# Autodesk Inventor assembly: RollerAssemblyBearing
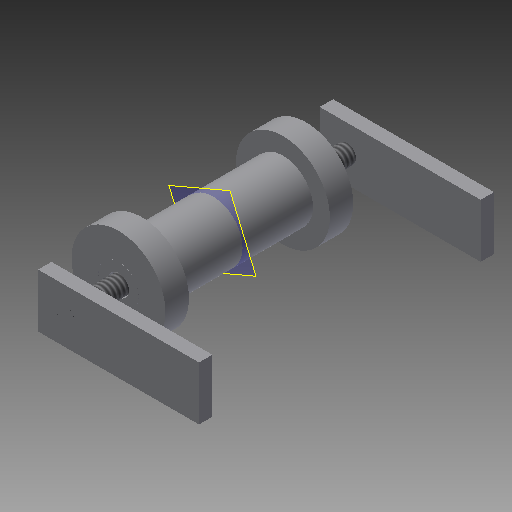
[picture p0: Inventor's stored thumbnail of the model, 512x512]
Saved by Autodesk Inventor 2018.3 (Build 223284000, 284)
## iProperties
Created: 2020-01-25
Part Number: RollerAssemblyBearing
Document SubType Name: Assembly
Designer: 22jungchan
Mass: 11.8553 g
Surface Area: 79.9251 cm^2
Volume: 11.8553 cm^3
Density: 1 g/cm^3
Author: 22jungchan
## Documents named in this file (5)
- C:\Users\22perngrac\Documents\GrabCAD\Infinite Recharge 2020\Build season\CLB_025_RollerAssembly(Bearing)S4.iam
- C:\Users\22perngrac\Documents\GrabCAD\Infinite Recharge 2020\Build season\CLB_016_RollerShaftS4.ipt
- C:\Users\22perngrac\Documents\GrabCAD\Infinite Recharge 2020\Build season\CLB_010_RollerSquareBracket.ipt
- C:\Users\22perngrac\Documents\GrabCAD\Infinite Recharge 2020\Build season\CLB_013_RollerSpacer2(Bearing)-S4.ipt
- C:\Users\22perngrac\Documents\GrabCAD\Infinite Recharge 2020\Build season\CLB_014_Bearing.ipt
## Components (6 placed, 4 different names)
1. CLB_016_RollerShaftS4:1 — Insert:1, Insert:4, Flush:4, Mate:4
2. CLB_010_RollerSquareBracket:3 — Insert:1, Flush:3
3. CLB_010_RollerSquareBracket:4 — Insert:4, Flush:3
4. CLB_013_RollerSpacer2(Bearing)-S4:1 — Mate:1, Flush:1, Flush:2, Mate:2, Mate:3, Flush:4, Mate:4
5. CLB_014_Bearing:3 — Flush:1, Mate:2
6. CLB_014_Bearing:4 — Mate:1, Flush:2, Mate:3
## Relationships (10: Mate 4, Flush 4, Insert 2)
- Insert:1: CLB_016_RollerShaftS4:1 ↔ CLB_010_RollerSquareBracket:3
- Insert:4: CLB_016_RollerShaftS4:1 ↔ CLB_010_RollerSquareBracket:4
- Mate:1: CLB_013_RollerSpacer2(Bearing)-S4:1 ↔ CLB_014_Bearing:4
- Flush:1: CLB_013_RollerSpacer2(Bearing)-S4:1 ↔ CLB_014_Bearing:3
- Flush:2: CLB_013_RollerSpacer2(Bearing)-S4:1 ↔ CLB_014_Bearing:4
- Mate:2: CLB_013_RollerSpacer2(Bearing)-S4:1 ↔ CLB_014_Bearing:3
- Mate:3: CLB_013_RollerSpacer2(Bearing)-S4:1 ↔ CLB_014_Bearing:4
- Flush:3: CLB_010_RollerSquareBracket:3 ↔ CLB_010_RollerSquareBracket:4
- Flush:4: CLB_016_RollerShaftS4:1 ↔ CLB_013_RollerSpacer2(Bearing)-S4:1
- Mate:4: CLB_016_RollerShaftS4:1 ↔ CLB_013_RollerSpacer2(Bearing)-S4:1
